# Autodesk Inventor assembly: Outer Channel
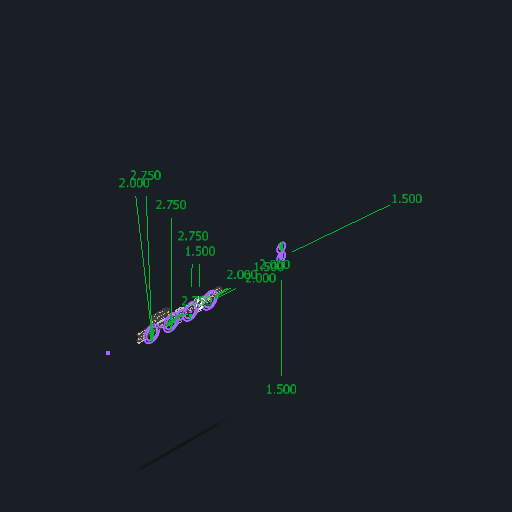
[picture p0: Inventor's stored thumbnail of the model, 512x512]
Saved by Autodesk Inventor 2025.1 (Build 291241000, 241)
## iProperties
Created: 2024-11-04
Part Number: Outer Channel
Document SubType Name: Assembly
Designer: avere
Author: avere
## Documents named in this file (27)
- C:\Users\avere\VEX\High Stakes\CAD\V3\Chassis\Drivebay Right\Outer Channel.iam
- C:\Users\avere\VEX\High Stakes\CAD\V3\Chassis\Drivebay Right\Alu C 1x2x1x30.ipt
- C:\Users\avere\VEX\High Stakes\CAD\V3\Chassis\Drivebay Right\Alu C 1x2x1x6.ipt
- C:\Users\avere\VEX\High Stakes\CAD\V3\Chassis\Drivebay Right\Bearing Flat.ipt
- C:\Users\avere\VEX\High Stakes\CAD\ROBOPROS-CAD-Inventor\Motion\Spacers\Spacer Nylon .500 OD\NSpacer White .500 OD x .250.ipt
- C:\Users\avere\VEX\High Stakes\CAD\ROBOPROS-CAD-Inventor\Motion\Spacers\Spacer Nylon .500 OD.ipt
- C:\Users\avere\VEX\High Stakes\CAD\V3\Chassis\Drivebay Right\Bearing Flat NScrew Slotted.iam
- C:\Users\avere\VEX\High Stakes\CAD\V3\Chassis\Drivebay Right\Bearing Flat NScrew Slotted Offset.iam
- C:\Users\avere\VEX\High Stakes\CAD\ROBOPROS-CAD-Inventor\Structure\Hardware\Screw Steel - Star\SScrew Star Smooth 1.750.ipt
- C:\Users\avere\VEX\High Stakes\CAD\ROBOPROS-CAD-Inventor\Structure\Hardware\Screw Steel - Star.ipt
- C:\Users\avere\VEX\High Stakes\CAD\ROBOPROS-CAD-Inventor\Motion\Spacers\Spacer Nylon .375 OD\NSpacer .375 OD x .875.ipt
- C:\Users\avere\VEX\High Stakes\CAD\ROBOPROS-CAD-Inventor\Motion\Spacers\Spacer Nylon .375 OD.ipt
- C:\Users\avere\VEX\High Stakes\CAD\V3\Chassis\Drivebay Right\Nut Nylon Thread-Forming.ipt
- C:\Users\avere\VEX\High Stakes\CAD\ROBOPROS-CAD-Inventor\Structure\Hardware\Screw Shoulder Robosource\SScrew Shoulder Smooth .375 x .12.ipt
- C:\Users\avere\VEX\High Stakes\CAD\ROBOPROS-CAD-Inventor\Structure\Hardware\Screw Shoulder Robosource.ipt
- C:\Users\avere\VEX\High Stakes\CAD\ROBOPROS-CAD-Inventor\Structure\Hardware\Screw Steel - Star\SScrew Star Smooth .250.ipt
- C:\Users\avere\VEX\High Stakes\CAD\V3\Chassis\Drivebay Right\Nylon Standoff .875.ipt
- C:\Users\avere\VEX\High Stakes\CAD\ROBOPROS-CAD-Inventor\Motion\Spacers\Spacer Nylon .375 OD\NSpacer .375 OD x .500.ipt
- C:\Users\avere\VEX\High Stakes\CAD\ROBOPROS-CAD-Inventor\Structure\Hardware\Nut Nylon\Nut Nylon - White.ipt
- C:\Users\avere\VEX\High Stakes\CAD\ROBOPROS-CAD-Inventor\Structure\Hardware\Nut Nylon.ipt
- C:\Users\avere\VEX\High Stakes\CAD\ROBOPROS-CAD-Inventor\Structure\Hardware\Screw Shoulder Robosource\SScrew Shoulder Smooth 2.000 x .04.ipt
- C:\Users\avere\VEX\High Stakes\CAD\V3\Chassis\Drivebay Right\Bearing Flat Low Profile 2-Hole.ipt
- C:\Users\avere\VEX\High Stakes\CAD\V3\Chassis\Drivebay Right\1-Post Hex Nut Retainer With Nylon Hardware.iam
- C:\Users\avere\VEX\High Stakes\CAD\ROBOPROS-CAD-Inventor\Motion\Spacers\Spacer Nylon .500 OD\NSpacer White .500 OD x .125.ipt
- C:\Users\avere\VEX\High Stakes\CAD\ROBOPROS-CAD-Inventor\Motion\Spacers\Washer Steel\SWasher .500 OD x .062500\SWasher .500 OD x .062500.ipt
- C:\Users\avere\VEX\High Stakes\CAD\ROBOPROS-CAD-Inventor\Motion\Spacers\Washer Steel\SWasher .500 OD x .062500.ipt
- C:\Users\avere\VEX\High Stakes\CAD\V3\Chassis\Drivebay Right\NScrew Slotted Threaded .500.ipt
## Components (56 placed, 20 different names)
1. Alu C 1x2x1x30:1 — Flush:2, Flush:3, Flush:1, Mate:19, Insert:58, Mate:3, Insert:12, Mate:21, Insert:62, Insert:63, Mate:18, Insert:57, Insert:65, Insert:61, Insert:60, Insert:66, Insert:45, Insert:44, Insert:46, Insert:47, Mate:15, Insert:50, Insert:55, Mate:17, Insert:56, Insert:67, Insert:68, Insert:69, Insert:76, Insert:77, Insert:75, Mate:25, Insert:74, Insert:79, Insert:80, Insert:78, Insert:49, Insert:51, Mate:16, Insert:52, Insert:53, Mate:17
2. Alu C 1x2x1x6:1 — Insert:64, Insert:32, Mate:12, Insert:37, Insert:38, Insert:39, Insert:81, Insert:82, Insert:83, Insert:84, Insert:85
3. Bearing Flat:1 — Mate:21, Insert:62, Insert:87
4. Bearing Flat:2 — Insert:63, Insert:20, Mate:22
5. NSpacer White .500 OD x .250:1 — Insert:64, Insert:20
6. Bearing Flat NScrew Slotted:1 [sub-assembly] — Mate:12, Insert:37
7. Bearing Flat NScrew Slotted Offset:1 [sub-assembly] — Mate:18, Insert:57
8. SScrew Star Smooth 1.750:1 — Insert:65, Mate:27
9. SScrew Star Smooth 1.750:2 — Insert:61
10. NSpacer .375 OD x .875:1 — Mate:22, Insert:60
11. NSpacer .375 OD x .875:2 — Insert:66
12. Nut Nylon Thread-Forming:1 — Insert:85
13. SScrew Shoulder Smooth .375 x .12:1 — Insert:84
14. SScrew Shoulder Smooth .375 x .12:2 — Insert:83
15. SScrew Star Smooth .250:3 — Insert:32
16. Nylon Standoff .875:1 — Mate:27, Insert:38
17. Nylon Standoff .875:2 — Insert:39
18. NSpacer .375 OD x .500:3 — Insert:54, Insert:51
19. NSpacer .375 OD x .500:4 — Insert:53, Insert:52
20. Nut Nylon - White:1 — Insert:45
21. Nut Nylon - White:2 — Insert:44
22. Nut Nylon - White:3 — Insert:46
23. Nut Nylon - White:4 — Insert:47
24. SScrew Shoulder Smooth 2.000 x .04:3 — Insert:53, Mate:16
25. SScrew Shoulder Smooth 2.000 x .04:4 — Insert:54
26. Bearing Flat Low Profile 2-Hole:1 — Insert:52, Insert:51, Mate:15, Insert:50
27. 1-Post Hex Nut Retainer With Nylon Hardware:1 [sub-assembly] — Mate:16, Insert:55
28. 1-Post Hex Nut Retainer With Nylon Hardware:2 [sub-assembly] — Mate:17, Insert:56
29. NSpacer .375 OD x .500:5 — Insert:73, Insert:70
30. NSpacer .375 OD x .500:6 — Insert:72, Insert:71
31. Nut Nylon - White:5 — Insert:76
32. Nut Nylon - White:6 — Insert:77
33. Nut Nylon - White:7 — Insert:75
34. SScrew Shoulder Smooth 2.000 x .04:5 — Insert:72, Mate:24
35. SScrew Shoulder Smooth 2.000 x .04:6 — Insert:73, Mate:15
36. Bearing Flat Low Profile 2-Hole:2 — Mate:25, Insert:74, Insert:71, Insert:70
37. 1-Post Hex Nut Retainer With Nylon Hardware:3 [sub-assembly] — Insert:79, Mate:24
38. 1-Post Hex Nut Retainer With Nylon Hardware:4 [sub-assembly] — Insert:80, Mate:15
39. Nut Nylon - White:8 — Insert:78
40. Nylon Standoff .875:3 — Insert:67
41. Nylon Standoff .875:4 — Insert:68
42. Nylon Standoff .875:5 — Insert:69
43. Nut Nylon Thread-Forming:2 — Insert:81
44. Nut Nylon Thread-Forming:3 — Insert:82
45. NSpacer White .500 OD x .125:2 — Insert:87, Insert:86
46. SWasher .500 OD x .062500:1 — Insert:86
47. Nylon Standoff .875:6 — Insert:49
48. Bearing Flat Low Profile 2-Hole:3 — Insert:51, Mate:16
49. NScrew Slotted Threaded .500:1 — Insert:52
50. Nut Nylon - White:9
51. Bearing Flat:3 — Insert:53, Mate:17
52. Bearing Flat NScrew Slotted:2 [sub-assembly] — Mate:3, Insert:12
53. Bearing Flat NScrew Slotted:4 [sub-assembly]
54. Bearing Flat NScrew Slotted:5 [sub-assembly]
55. Bearing Flat NScrew Slotted:3 [sub-assembly] — Mate:19, Insert:58
56. Bearing Flat NScrew Slotted:6 [sub-assembly]
## Component patterns: (3 elements, first: Bearing Flat NScrew Slotted:2), (2 elements, first: Bearing Flat NScrew Slotted:3)
## Relationships (70: Insert 52, Mate 16, Flush 2)
- Flush:2 (-38.1 mm): Alu C 1x2x1x30:1
- Flush:3 (-7.9375 mm): Alu C 1x2x1x30:1
- Flush:1 [Mate] (-190.5 mm): Alu C 1x2x1x30:1
- Mate:19: Alu C 1x2x1x30:1 ↔ Bearing Flat NScrew Slotted:3
- Insert:58: Alu C 1x2x1x30:1 ↔ Bearing Flat NScrew Slotted:3
- Mate:3: Alu C 1x2x1x30:1 ↔ Bearing Flat NScrew Slotted:2
- Insert:12: Alu C 1x2x1x30:1 ↔ Bearing Flat NScrew Slotted:2
- Mate:21: Alu C 1x2x1x30:1 ↔ Bearing Flat:1
- Insert:62: Alu C 1x2x1x30:1 ↔ Bearing Flat:1
- Insert:63: Alu C 1x2x1x30:1 ↔ Bearing Flat:2
- Insert:64: Alu C 1x2x1x6:1 ↔ NSpacer White .500 OD x .250:1
- Insert:20: Bearing Flat:2 ↔ NSpacer White .500 OD x .250:1
- Mate:18: Alu C 1x2x1x30:1 ↔ Bearing Flat NScrew Slotted Offset:1
- Insert:57: Alu C 1x2x1x30:1 ↔ Bearing Flat NScrew Slotted Offset:1
- Insert:65: Alu C 1x2x1x30:1 ↔ SScrew Star Smooth 1.750:1
- Insert:61: Alu C 1x2x1x30:1 ↔ SScrew Star Smooth 1.750:2
- Insert:32: Alu C 1x2x1x6:1 ↔ SScrew Star Smooth .250:3
- Mate:22: Bearing Flat:2 ↔ NSpacer .375 OD x .875:1
- Insert:60: Alu C 1x2x1x30:1 ↔ NSpacer .375 OD x .875:1
- Insert:66: Alu C 1x2x1x30:1 ↔ NSpacer .375 OD x .875:2
- Mate:12: Alu C 1x2x1x6:1 ↔ Bearing Flat NScrew Slotted:1
- Insert:37: Alu C 1x2x1x6:1 ↔ Bearing Flat NScrew Slotted:1
- Mate:27: SScrew Star Smooth 1.750:1 ↔ Nylon Standoff .875:1
- Insert:38: Alu C 1x2x1x6:1 ↔ Nylon Standoff .875:1
- Insert:39: Alu C 1x2x1x6:1 ↔ Nylon Standoff .875:2
- Insert:45: Alu C 1x2x1x30:1 ↔ Nut Nylon - White:1
- Insert:44: Alu C 1x2x1x30:1 ↔ Nut Nylon - White:2
- Insert:46: Alu C 1x2x1x30:1 ↔ Nut Nylon - White:3
- Insert:47: Alu C 1x2x1x30:1 ↔ Nut Nylon - White:4
- Insert:53 (1.5875 mm): NSpacer .375 OD x .500:4 ↔ SScrew Shoulder Smooth 2.000 x .04:3
- Insert:54 (1.5875 mm): NSpacer .375 OD x .500:3 ↔ SScrew Shoulder Smooth 2.000 x .04:4
- Insert:52 (1.27 mm): NSpacer .375 OD x .500:4 ↔ Bearing Flat Low Profile 2-Hole:1
- Insert:51 (1.27 mm): NSpacer .375 OD x .500:3 ↔ Bearing Flat Low Profile 2-Hole:1
- Mate:15: Alu C 1x2x1x30:1 ↔ Bearing Flat Low Profile 2-Hole:1
- Insert:50: Alu C 1x2x1x30:1 ↔ Bearing Flat Low Profile 2-Hole:1
- Mate:16: SScrew Shoulder Smooth 2.000 x .04:3 ↔ 1-Post Hex Nut Retainer With Nylon Hardware:1
- Insert:55: Alu C 1x2x1x30:1 ↔ 1-Post Hex Nut Retainer With Nylon Hardware:1
- Mate:17: Alu C 1x2x1x30:1 ↔ 1-Post Hex Nut Retainer With Nylon Hardware:2
- Insert:56: Alu C 1x2x1x30:1 ↔ 1-Post Hex Nut Retainer With Nylon Hardware:2
- Insert:67: Alu C 1x2x1x30:1 ↔ Nylon Standoff .875:3
- Insert:68: Alu C 1x2x1x30:1 ↔ Nylon Standoff .875:4
- Insert:69: Alu C 1x2x1x30:1 ↔ Nylon Standoff .875:5
- Insert:76: Alu C 1x2x1x30:1 ↔ Nut Nylon - White:5
- Insert:77: Alu C 1x2x1x30:1 ↔ Nut Nylon - White:6
- Insert:75: Alu C 1x2x1x30:1 ↔ Nut Nylon - White:7
- Insert:72 (1.5875 mm): NSpacer .375 OD x .500:6 ↔ SScrew Shoulder Smooth 2.000 x .04:5
- Insert:73 (1.5875 mm): NSpacer .375 OD x .500:5 ↔ SScrew Shoulder Smooth 2.000 x .04:6
- Mate:25: Alu C 1x2x1x30:1 ↔ Bearing Flat Low Profile 2-Hole:2
- Insert:74: Alu C 1x2x1x30:1 ↔ Bearing Flat Low Profile 2-Hole:2
- Insert:71 (1.27 mm): NSpacer .375 OD x .500:6 ↔ Bearing Flat Low Profile 2-Hole:2
- Insert:70 (1.27 mm): NSpacer .375 OD x .500:5 ↔ Bearing Flat Low Profile 2-Hole:2
- Insert:79: Alu C 1x2x1x30:1 ↔ 1-Post Hex Nut Retainer With Nylon Hardware:3
- Mate:24: SScrew Shoulder Smooth 2.000 x .04:5 ↔ 1-Post Hex Nut Retainer With Nylon Hardware:3
- Insert:80: Alu C 1x2x1x30:1 ↔ 1-Post Hex Nut Retainer With Nylon Hardware:4
- Insert:78: Alu C 1x2x1x30:1 ↔ Nut Nylon - White:8
- Insert:81: Alu C 1x2x1x6:1 ↔ Nut Nylon Thread-Forming:2
- Insert:82: Alu C 1x2x1x6:1 ↔ Nut Nylon Thread-Forming:3
- Insert:83 (1.5875 mm): Alu C 1x2x1x6:1 ↔ SScrew Shoulder Smooth .375 x .12:2
- Insert:84: Alu C 1x2x1x6:1 ↔ SScrew Shoulder Smooth .375 x .12:1
- Insert:85 (1.5875 mm): Alu C 1x2x1x6:1 ↔ Nut Nylon Thread-Forming:1
- Insert:87: Bearing Flat:1 ↔ NSpacer White .500 OD x .125:2
- Insert:86: NSpacer White .500 OD x .125:2 ↔ SWasher .500 OD x .062500:1
- Mate:15: SScrew Shoulder Smooth 2.000 x .04:6 ↔ 1-Post Hex Nut Retainer With Nylon Hardware:4
- Insert:49: Alu C 1x2x1x30:1 ↔ Nylon Standoff .875:6
- [Insert] (1.27 mm): Bearing Flat Low Profile 2-Hole:3 ↔ Nut Nylon - White:9
- Insert:51: Alu C 1x2x1x30:1 ↔ Bearing Flat Low Profile 2-Hole:3
- Mate:16: Alu C 1x2x1x30:1 ↔ Bearing Flat Low Profile 2-Hole:3
- Insert:52: Alu C 1x2x1x30:1 ↔ NScrew Slotted Threaded .500:1
- Insert:53: Alu C 1x2x1x30:1 ↔ Bearing Flat:3
- Mate:17: Alu C 1x2x1x30:1 ↔ Bearing Flat:3
## Named parameters: d78_d53 = 1.27 mm
